# Autodesk Inventor assembly: ASY ДМФ 0100 Барабан v2.1
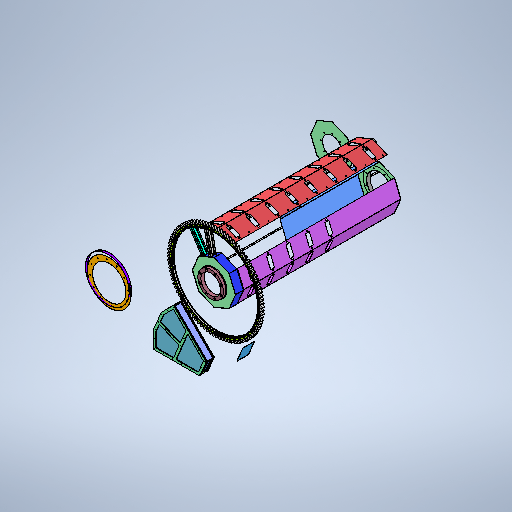
[picture p0: Inventor's stored thumbnail of the model, 512x512]
Saved by Autodesk Inventor 2025 (Build 290162010, 162A)
## iProperties
Created: 2024-04-28
Part Number: ASY ДМФ 0100 Барабан v2.1
Document SubType Name: Assembly
Designer: pokla
Author: pokla
## Documents named in this file (21)
- C:\Users\admin\Yandex.Disk\home pc\Inventor\DMF-Disk-Micro-Filter\Барабан v2.1\ASY ДМФ 0100 Барабан v2.1.iam
- C:\Users\admin\Yandex.Disk\home pc\Inventor\DMF-Disk-Micro-Filter\Барабан v2.1\DMF 01 21 Барабан торец НОС v2.1.ipt
- C:\Users\admin\Yandex.Disk\home pc\Inventor\DMF-Disk-Micro-Filter\Барабан v2.1\DMF 01 13 Барабан Лист лев брт v2.1.ipt
- C:\Users\admin\Yandex.Disk\home pc\Inventor\DMF-Disk-Micro-Filter\Барабан v2.1\DMF 01 14 Барабан Лист прав брт v2.1.ipt
- C:\Users\admin\Yandex.Disk\home pc\Inventor\DMF-Disk-Micro-Filter\Барабан v2.1\DMF 01 31 Барабан Опорное кольцо НОС v2.1.ipt
- C:\Users\admin\Yandex.Disk\home pc\Inventor\DMF-Disk-Micro-Filter\Барабан v2.1\DMF 01 17 опора крышки v2.1.ipt
- C:\Users\admin\Yandex.Disk\home pc\Inventor\DMF-Disk-Micro-Filter\Барабан v2.1\DMF 000 размеры v2.1.ipt
- C:\Users\admin\Yandex.Disk\home pc\Inventor\DMF-Disk-Micro-Filter\Барабан v2.1\DMF 01 12 Барабан усилитель v2.1.ipt
- C:\Users\admin\Yandex.Disk\home pc\Inventor\DMF-Disk-Micro-Filter\Барабан v2.1\ASY DMF 010 cap v2.1.iam
- C:\Users\admin\Yandex.Disk\home pc\Inventor\DMF-Disk-Micro-Filter\Барабан v2.1\DMF 01 32 Барабан Опорное кольцо КОРМА v2.1.ipt
- C:\Users\admin\Yandex.Disk\home pc\Inventor\DMF-Disk-Micro-Filter\Барабан v2.1\DMF 01 22 Барабан торец КОРМА v2.1.ipt
- C:\Users\admin\Yandex.Disk\home pc\Inventor\DMF-Disk-Micro-Filter\Барабан v2.1\ASY DMF filter package v2.1.iam
- C:\Users\admin\Yandex.Disk\home pc\Inventor\DMF-Disk-Micro-Filter\Барабан v2.1\DMF 01 21 cylinder butt end nose.ipt
- C:\Users\admin\Yandex.Disk\home pc\Inventor\DMF-Disk-Micro-Filter\Барабан v2.1\DMF 2.1 01 42 Gear way 2.ipt
- C:\Users\admin\Yandex.Disk\home pc\Inventor\DMF-Disk-Micro-Filter\Барабан v2.1\DMF 2.1 01 43 Gear rim 3.ipt
- C:\Users\admin\Yandex.Disk\home pc\Inventor\DMF-Disk-Micro-Filter\Барабан v2.1\DMF 2.1 01 44 Gear rim 4.ipt
- C:\Users\admin\Yandex.Disk\home pc\Inventor\DMF-Disk-Micro-Filter\Барабан v2.1\DMF 2.1 01 45 Gear ring 5.ipt
- C:\Users\admin\Yandex.Disk\home pc\Inventor\DMF-Disk-Micro-Filter\Барабан v2.1\DMF 2.1 01 46 Gear axis wheel 6.ipt
- C:\Users\admin\Yandex.Disk\home pc\Inventor\DMF-Disk-Micro-Filter\Барабан v2.1\DMF 01 13 Барабан усилитель v2.1.ipt
- C:\Users\admin\Yandex.Disk\home pc\Inventor\DMF-Disk-Micro-Filter\шестерни 06.09.2025\DMF sector big gear 2.1.ipt
- C:\Users\admin\Yandex.Disk\home pc\Inventor\DMF-Disk-Micro-Filter\Барабан v2.1\DMF 01 15 drum sheet 1.ipt
## Components (80 placed, 24 different names)
1. DMF 000 размеры v2.1.ipt:1
2. DMF 01 21 Барабан торец НОС v2.1.ipt:1 — Rigid:45, Rigid:46, Flush:21
3. DMF 01 31 Барабан Опорное кольцо НОС v2.1.ipt:1
4. DMF 01 32 Барабан Опорное кольцо КОРМА v2.1.ipt:1 — Rigid:20
5. DMF 01 22 Барабан торец КОРМА v2.1.ipt:1 — Flush:13, Mate:18, Rigid:20, Rigid:47
6. DMF 01 13 Барабан Лист лев брт v2.1.ipt:1 — Flush:13, Mate:18, Mate:29
7. DMF 01 14 Барабан Лист прав брт v2.1.ipt:1 — Rigid:47
8. DMF 01 17 опора крышки v2.1.ipt:1
9. DMF 01 17 опора крышки v2.1.ipt:2
10. ASY DMF 010 cap v2.1.iam:1 [sub-assembly]
11. ASY DMF filter package v2.1.iam:1 [sub-assembly]
12. DMF 01 21 cylinder butt end nose.ipt:1 — Mate:29
13. DMF 2.1 01 45 Gear ring 5.ipt:1
14. DMF 2.1 01 46 Gear axis wheel 6.ipt:1
15. DMF 2.1 01 44 Gear rim 4.ipt:1 — Rigid:39, Rigid:40, Rigid:41
16. DMF 2.1 01 43 Gear rim 3.ipt:2 — Rigid:24, Rigid:35
17. DMF 2.1 01 43 Gear rim 3.ipt:1 — Rigid:24
18. DMF 2.1 01 42 Gear way 2.ipt:1
19. DMF 2.1 01 43 Gear rim 3:3 — Rigid:35, Rigid:36, Rigid:39
20. DMF 2.1 01 43 Gear rim 3:4
21. DMF 2.1 01 43 Gear rim 3:5 — Rigid:36, Rigid:38, Flush:18, Mate:33, Mate:34, Tangent:1
22. DMF 2.1 01 43 Gear rim 3:6 — Rigid:42
23. DMF 2.1 01 43 Gear rim 3:7 — Rigid:38
24. DMF 2.1 01 43 Gear rim 3:8
25. DMF 2.1 01 44 Gear rim 4:2 — Rigid:40
26. DMF 2.1 01 44 Gear rim 4:3 — Rigid:41
27. DMF 01 13 Барабан усилитель v2.1.ipt:1 — Rigid:43, Flush:19
28. DMF 01 12 Барабан усилитель v2.1:50 — Flush:18, Mate:33, Mate:34, Rigid:43, Flush:20, Mate:35, Flush:21
29. ДМФ 01 13 Барабан усилитель v2.0:2 — Tangent:1
30. DMF 01 12 Барабан усилитель v2.1:51 — Flush:19, Flush:20
31. DMF 01 15 drum sheet 1:1 — Rigid:46
32. DMF 01 15 drum sheet 1:2 — Rigid:45, Mate:35
33. DMF sector big gear 2.1.ipt:1 — Rigid:42
34. DMF sector big gear 2.1:2
35. DMF sector big gear 2.1:3
36. DMF sector big gear 2.1:4
37. DMF sector big gear 2.1:5
38. DMF sector big gear 2.1:6
39. DMF sector big gear 2.1:7
40. DMF sector big gear 2.1:8
41. DMF sector big gear 2.1:9
42. DMF sector big gear 2.1:10
43. DMF sector big gear 2.1:11
44. DMF sector big gear 2.1:12
45. DMF sector big gear 2.1:13
46. DMF sector big gear 2.1:14
47. DMF sector big gear 2.1:15
48. DMF sector big gear 2.1:16
49. DMF sector big gear 2.1:17
50. DMF sector big gear 2.1:18
51. DMF sector big gear 2.1:19
52. DMF sector big gear 2.1:20
53. DMF sector big gear 2.1:21
54. DMF sector big gear 2.1:22
55. DMF sector big gear 2.1:23
56. DMF sector big gear 2.1:24
57. DMF sector big gear 2.1:25
58. DMF sector big gear 2.1:26
59. DMF sector big gear 2.1:27
60. DMF sector big gear 2.1:28
61. DMF sector big gear 2.1:29
62. DMF sector big gear 2.1:30
63. DMF sector big gear 2.1:31
64. DMF sector big gear 2.1:32
65. DMF sector big gear 2.1:33
66. DMF sector big gear 2.1:34
67. DMF sector big gear 2.1:35
68. DMF sector big gear 2.1:36
69. DMF sector big gear 2.1:37
70. DMF sector big gear 2.1:38
71. DMF sector big gear 2.1:39
72. DMF sector big gear 2.1:40
73. DMF sector big gear 2.1:41
74. DMF sector big gear 2.1:42
75. DMF sector big gear 2.1:43
76. DMF sector big gear 2.1:44
77. DMF sector big gear 2.1:45
78. DMF sector big gear 2.1:46
79. DMF sector big gear 2.1:47
80. DMF sector big gear 2.1:48
## Component patterns: (48 elements, first: DMF sector big gear 2.1.ipt:1)
## Relationships (28: WeldJoint 17, Flush 5, Mate 5, Tangent 1)
- Flush:13: DMF 01 22 Барабан торец КОРМА v2.1.ipt:1 ↔ DMF 01 13 Барабан Лист лев брт v2.1.ipt:1
- Mate:18: DMF 01 22 Барабан торец КОРМА v2.1.ipt:1 ↔ DMF 01 13 Барабан Лист лев брт v2.1.ipt:1
- Mate:29: DMF 01 13 Барабан Лист лев брт v2.1.ipt:1 ↔ DMF 01 21 cylinder butt end nose.ipt:1
- Rigid:20 [WeldJoint]: DMF 01 32 Барабан Опорное кольцо КОРМА v2.1.ipt:1 ↔ DMF 01 22 Барабан торец КОРМА v2.1.ipt:1
- Rigid:24 [WeldJoint] (25 mm): DMF 2.1 01 43 Gear rim 3.ipt:2 ↔ DMF 2.1 01 43 Gear rim 3.ipt:1
- [WeldJoint] (25 mm): DMF 2.1 01 43 Gear rim 3:3 ↔ DMF 2.1 01 43 Gear rim 3:4
- [WeldJoint] (25 mm): DMF 2.1 01 43 Gear rim 3:5 ↔ DMF 2.1 01 43 Gear rim 3:6
- Rigid:35 [WeldJoint]: DMF 2.1 01 43 Gear rim 3.ipt:2 ↔ DMF 2.1 01 43 Gear rim 3:3
- Rigid:36 [WeldJoint]: DMF 2.1 01 43 Gear rim 3:3 ↔ DMF 2.1 01 43 Gear rim 3:5
- [WeldJoint] (25 mm): DMF 2.1 01 43 Gear rim 3:7 ↔ DMF 2.1 01 43 Gear rim 3:8
- Rigid:38 [WeldJoint]: DMF 2.1 01 43 Gear rim 3:5 ↔ DMF 2.1 01 43 Gear rim 3:7
- Rigid:39 [WeldJoint]: DMF 2.1 01 44 Gear rim 4.ipt:1 ↔ DMF 2.1 01 43 Gear rim 3:3
- Rigid:40 [WeldJoint]: DMF 2.1 01 44 Gear rim 4.ipt:1 ↔ DMF 2.1 01 44 Gear rim 4:2
- Rigid:41 [WeldJoint]: DMF 2.1 01 44 Gear rim 4.ipt:1 ↔ DMF 2.1 01 44 Gear rim 4:3
- Rigid:42 [WeldJoint]: DMF 2.1 01 43 Gear rim 3:6 ↔ DMF sector big gear 2.1.ipt:1
- Flush:18: DMF 2.1 01 43 Gear rim 3:5 ↔ DMF 01 12 Барабан усилитель v2.1:50
- Mate:33: DMF 2.1 01 43 Gear rim 3:5 ↔ DMF 01 12 Барабан усилитель v2.1:50
- Mate:34: DMF 2.1 01 43 Gear rim 3:5 ↔ DMF 01 12 Барабан усилитель v2.1:50
- Rigid:43 [WeldJoint]: DMF 01 13 Барабан усилитель v2.1.ipt:1 ↔ DMF 01 12 Барабан усилитель v2.1:50
- [WeldJoint]: ДМФ 01 13 Барабан усилитель v2.0:2 ↔ DMF 01 12 Барабан усилитель v2.1:51
- Flush:19: DMF 01 13 Барабан усилитель v2.1.ipt:1 ↔ DMF 01 12 Барабан усилитель v2.1:51
- Flush:20: DMF 01 12 Барабан усилитель v2.1:50 ↔ DMF 01 12 Барабан усилитель v2.1:51
- Tangent:1: DMF 2.1 01 43 Gear rim 3:5 ↔ ДМФ 01 13 Барабан усилитель v2.0:2
- Rigid:45 [WeldJoint]: DMF 01 21 Барабан торец НОС v2.1.ipt:1 ↔ DMF 01 15 drum sheet 1:2
- Rigid:46 [WeldJoint]: DMF 01 21 Барабан торец НОС v2.1.ipt:1 ↔ DMF 01 15 drum sheet 1:1
- Mate:35: DMF 01 12 Барабан усилитель v2.1:50 ↔ DMF 01 15 drum sheet 1:2
- Flush:21 (10 mm): DMF 01 21 Барабан торец НОС v2.1.ipt:1 ↔ DMF 01 12 Барабан усилитель v2.1:50
- Rigid:47 [WeldJoint]: DMF 01 22 Барабан торец КОРМА v2.1.ipt:1 ↔ DMF 01 14 Барабан Лист прав брт v2.1.ipt:1
## Named parameters: d314_d251 = 25 mm, d315_d251 = 25 mm, d318_d251 = 25 mm, d336_d335 = 0 mm
